# Autodesk Inventor assembly: 1 Wheel Board
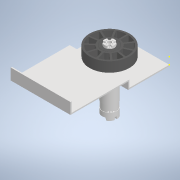
[picture p0: Inventor's stored thumbnail of the model, 180x180]
Saved by Autodesk Inventor 2020.3 (Build 243373010, 373A)
## iProperties
Created: 2020-10-01
Part Number: 1 Wheel Board
Document SubType Name: Assembly
Designer: Owner
Author: Owner
## Documents named in this file (7)
- C:\Users\Owner\Documents\GitHub\CAD-2021-Ultimate_Goal\Shooter\1 Wheel Board.iam
- C:\Users\Owner\Documents\GitHub\CAD-2021-Ultimate_Goal\Shooter\Single Sided board.ipt
- C:\Users\Owner\Documents\GitHub\CAD-2021-Ultimate_Goal\ServoCity\1206-0016-0004 assembly.iam
- C:\Users\Owner\Documents\GitHub\CAD-2021-Ultimate_Goal\GoBilda\5202-0002-0003 part.ipt
- C:\Users\Owner\Documents\GitHub\CAD-2021-Ultimate_Goal\ServoCity\545456.ipt
- C:\Users\Owner\Documents\GitHub\CAD-2021-Ultimate_Goal\ServoCity\545636 assembly.ipt
- C:\Users\Owner\Documents\GitHub\CAD-2021-Ultimate_Goal\AndyMark\am-3563 4IN 8mm Round Compliant Wheel REV2.ipt
## Components (7 placed, 6 different names)
1. Single Sided board:1 — Mate:1, Mate:2, Mate:3, Mate:4, Mate:5, Mate:6
2. 1206-0016-0004 assembly:1 [sub-assembly] — Mate:1, Mate:2, Mate:16, Mate:17
3. 5202-0002-0003 part:1 — Mate:3, Mate:4, Mate:5, Mate:6
4. 545456:1 — Mate:7, Mate:8, Mate:9, Mate:10, Mate:11, Mate:12
5. 545456:2 — Mate:13, Mate:14, Mate:15, Mate:18
6. 545636 assembly:1 — Mate:10, Mate:11, Mate:12, Mate:16, Mate:17
7. am-3563 4IN 8mm Round Compliant Wheel REV2:1 — Mate:7, Mate:8, Mate:9, Mate:13, Mate:14, Mate:15, Mate:18
## Relationships (18: Mate 18)
- Mate:1: Single Sided board:1 ↔ 1206-0016-0004 assembly:1
- Mate:2: Single Sided board:1 ↔ 1206-0016-0004 assembly:1
- Mate:3: Single Sided board:1 ↔ 5202-0002-0003 part:1
- Mate:4: Single Sided board:1 ↔ 5202-0002-0003 part:1
- Mate:5: Single Sided board:1 ↔ 5202-0002-0003 part:1
- Mate:6: Single Sided board:1 ↔ 5202-0002-0003 part:1
- Mate:7: 545456:1 ↔ am-3563 4IN 8mm Round Compliant Wheel REV2:1
- Mate:8: 545456:1 ↔ am-3563 4IN 8mm Round Compliant Wheel REV2:1
- Mate:9: 545456:1 ↔ am-3563 4IN 8mm Round Compliant Wheel REV2:1
- Mate:10: 545456:1 ↔ 545636 assembly:1
- Mate:11: 545456:1 ↔ 545636 assembly:1
- Mate:12: 545456:1 ↔ 545636 assembly:1
- Mate:13: 545456:2 ↔ am-3563 4IN 8mm Round Compliant Wheel REV2:1
- Mate:14: 545456:2 ↔ am-3563 4IN 8mm Round Compliant Wheel REV2:1
- Mate:15: 545456:2 ↔ am-3563 4IN 8mm Round Compliant Wheel REV2:1
- Mate:16: 1206-0016-0004 assembly:1 ↔ 545636 assembly:1
- Mate:17: 1206-0016-0004 assembly:1 ↔ 545636 assembly:1
- Mate:18: 545456:2 ↔ am-3563 4IN 8mm Round Compliant Wheel REV2:1
